# Autodesk Inventor assembly: printer_larger
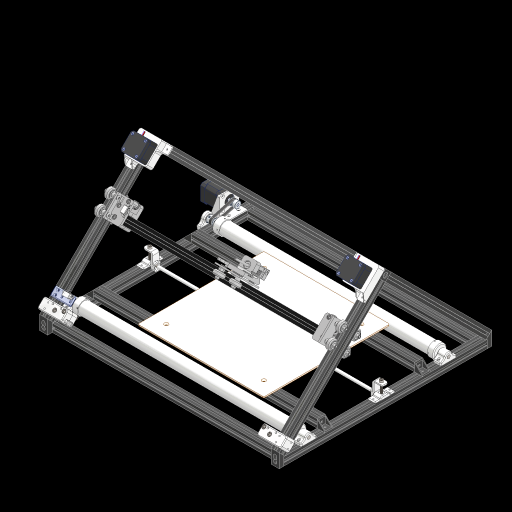
[picture p0: Inventor's stored thumbnail of the model, 512x512]
Saved by Autodesk Inventor 2023 (Build 270158000, 158)
## iProperties
Created: 2021-08-14
Part Number: printer_larger
Description: STEP AP214
Document SubType Name: Assembly
Designer: tandu
Sending System: SolidWorks 2020
Preprocessor: SwSTEP 2.0
Title: printer_larger.STEP
Revision Number: ANY
## Documents named in this file (38)
- C:\Users\tandu\Documents\GrabCAD\Custom Conveyor Belt 3D Printer\V1\Assembly.iam
- C:\Users\tandu\Documents\GrabCAD\Custom Conveyor Belt 3D Printer\V1\Parts\Frame\printer_largeeeFrame.iam
- C:\Users\tandu\Documents\GrabCAD\Custom Conveyor Belt 3D Printer\V1\Parts\printer_largeeeNEMA17_17HS19-2004S1_Stepperonline___ _________.ipt
- C:\Users\tandu\Documents\GrabCAD\Custom Conveyor Belt 3D Printer\V1\Parts\printer_largeeetensioner_mount.ipt
- C:\Users\tandu\Documents\GrabCAD\Custom Conveyor Belt 3D Printer\V1\Parts\printer_largeee5mm_roller_shaft.ipt
- C:\Users\tandu\Documents\GrabCAD\Custom Conveyor Belt 3D Printer\V1\Parts\printer_largeee330mm_cf_tube_thin.ipt
- C:\Users\tandu\Documents\GrabCAD\Custom Conveyor Belt 3D Printer\V1\Parts\printer_largeee605_bearing.ipt
- C:\Users\tandu\Documents\GrabCAD\Custom Conveyor Belt 3D Printer\V1\Parts\printer_largeeetube_mount_motor_side.ipt
- C:\Users\tandu\Documents\GrabCAD\Custom Conveyor Belt 3D Printer\V1\Parts\printer_largeeeGT2_20T_____________1.ipt
- C:\Users\tandu\Documents\GrabCAD\Custom Conveyor Belt 3D Printer\V1\Parts\printer_largeeeflange_coupling.ipt
- C:\Users\tandu\Documents\GrabCAD\Custom Conveyor Belt 3D Printer\V1\Parts\printer_largeeetube_holder_motor_side.ipt
- C:\Users\tandu\Documents\GrabCAD\Custom Conveyor Belt 3D Printer\V1\Parts\printer_largeeebelt_motor_mount.ipt
- C:\Users\tandu\Documents\GrabCAD\Custom Conveyor Belt 3D Printer\V1\Parts\printer_largeee330mm_cf_tube.ipt
- C:\Users\tandu\Documents\GrabCAD\Custom Conveyor Belt 3D Printer\V1\Parts\Build Plate\printer_largeeebed_mount_bracket.ipt
- C:\Users\tandu\Documents\GrabCAD\Custom Conveyor Belt 3D Printer\V1\Parts\printer_largeeetube_holder.ipt
- C:\Users\tandu\Documents\GrabCAD\Custom Conveyor Belt 3D Printer\V1\Parts\printer_largeeetube_mount.ipt
- C:\Users\tandu\Documents\GrabCAD\Custom Conveyor Belt 3D Printer\V1\Parts\printer_largeeeroller_rod.ipt
- C:\Users\tandu\Documents\GrabCAD\Custom Conveyor Belt 3D Printer\V1\Parts\printer_largeeeramp_mount.ipt
- C:\Users\tandu\Documents\GrabCAD\Custom Conveyor Belt 3D Printer\V1\Parts\Build Plate\printer_largeeebed_Predeterminado.ipt
- C:\Users\tandu\Documents\GrabCAD\Custom Conveyor Belt 3D Printer\V1\Parts\printer_largeeeBelt2-2987^printer_larger.ipt
- C:\Users\tandu\Documents\GrabCAD\Custom Conveyor Belt 3D Printer\V1\Parts\printer_largeeeF695 Bearing.step.ipt
- C:\Users\tandu\Documents\GrabCAD\Custom Conveyor Belt 3D Printer\V1\Parts\printer_largeeeleft_motor_mount.ipt
- C:\Users\tandu\Documents\GrabCAD\Custom Conveyor Belt 3D Printer\V1\Parts\printer_largeeeM5x40.ipt
- C:\Users\tandu\Documents\GrabCAD\Custom Conveyor Belt 3D Printer\V1\Parts\printer_largeeeright_motor_mount.ipt
- C:\Users\tandu\Documents\GrabCAD\Custom Conveyor Belt 3D Printer\V1\Parts\Gantry (Includes extruder folder)\printer_largeeegantry_idler_left.ipt
- C:\Users\tandu\Documents\GrabCAD\Custom Conveyor Belt 3D Printer\V1\Parts\Gantry (Includes extruder folder)\printer_largeeegantry_idler_right.ipt
- C:\Users\tandu\Documents\GrabCAD\Custom Conveyor Belt 3D Printer\V1\Parts\Gantry (Includes extruder folder)\printer_largeeegantry_idler_left_top.ipt
- C:\Users\tandu\Documents\GrabCAD\Custom Conveyor Belt 3D Printer\V1\Parts\Gantry (Includes extruder folder)\printer_largeeegantry_idler_right_top.ipt
- C:\Users\tandu\Documents\GrabCAD\Custom Conveyor Belt 3D Printer\V1\Parts\printer_largeeetensioner_mount_mount.ipt
- C:\Users\tandu\Documents\GrabCAD\Custom Conveyor Belt 3D Printer\V1\Parts\printer_largeeeM5x30.ipt
- C:\Users\tandu\Documents\GrabCAD\Custom Conveyor Belt 3D Printer\V1\Parts\printer_largeeey_switch_mount.ipt
- C:\Users\tandu\Documents\GrabCAD\Custom Conveyor Belt 3D Printer\V1\Parts\printer_largeeelimit_switch_cover_y.ipt
- C:\Users\tandu\Documents\GrabCAD\Custom Conveyor Belt 3D Printer\V1\Parts\printer_largeeeMicroswitch2.step_1.iam
- C:\Users\tandu\Documents\GrabCAD\Custom Conveyor Belt 3D Printer\V1\Parts\printer_largeeebearing_spacer.ipt
- C:\Users\tandu\Documents\GrabCAD\Custom Conveyor Belt 3D Printer\V1\Parts\Gantry (Includes extruder folder)\LeftGantryMount.iam
- C:\Users\tandu\Documents\GrabCAD\Custom Conveyor Belt 3D Printer\V1\Parts\Gantry (Includes extruder folder)\RightGantryMount.iam
- C:\Users\tandu\Documents\GrabCAD\Custom Conveyor Belt 3D Printer\V1\Parts\Gantry (Includes extruder folder)\Extruder\RollerVersionExtruder.iam
- C:\Users\tandu\Documents\GrabCAD\Custom Conveyor Belt 3D Printer\V1\Parts\Frame\Width Extrusion.ipt
## Components (70 placed, 69 different names)
1. Frame_1 [sub-assembly] — Tangent:1, Tangent:2, Mate:15, Angle:1, Symmetry:1, Flush:18, Mate:18, Flush:19, Mate:19, Flush:20, Flush:21, Mate:20, Mate:21, Mate:22, Mate:23, Flush:22, Flush:23, Mate:28, Mate:32, Flush:24, Flush:25, Mate:33, Mate:34, Flush:36, Flush:38, Mate:35, Angle:2, Mate:37, Mate:38, Mate:40, Flush:41, Angle:3, Mate:41, Flush:42, Mate:43, Flush:44, Mate:48, Flush:45, Flush:46, Flush:47, Mate:53, Mate:54, Mate:55, Mate:56, Mate:57, Flush:51, Flush:52, Mate:58
2. ramp_mount_34 — Flush:52, Mate:58
3. ramp_mount_35 — Mate:57, Flush:51
4. bearing_spacer_96 — Insert:32, Insert:33
5. bearing_spacer_95 — Insert:39, Insert:40
6. F695 Bearing.step_44 — Insert:33, Insert:34
7. F695 Bearing.step_45 — Insert:34
8. gantry_idler_left_59 — Insert:37, Flush:48
9. gantry_idler_right_60 — Insert:45, Flush:50
10. F695 Bearing.step_61 — Insert:40, Insert:41
11. F695 Bearing.step_62 — Insert:41
12. F695 Bearing.step_63 — Insert:38, Insert:39
13. F695 Bearing.step_64 — Insert:31, Insert:32
14. F695 Bearing.step_65 — Insert:30, Insert:31
15. F695 Bearing.step_66 — Insert:38, Insert:42
16. gantry_idler_left_top_71 — Flush:47, Mate:53, Mate:54, Insert:30, Insert:35, Insert:36, Insert:37, Flush:48, Flush:49
17. gantry_idler_right_top_72 — Flush:49, Mate:55, Mate:56, Insert:42, Insert:43, Insert:44, Insert:45, Flush:50
18. M5x40_76 — Insert:36
19. M5x40_80 — Insert:35
20. M5x40_81 — Insert:44
21. M5x40_82 — Insert:43
22. LeftGantryMount:1 [sub-assembly] — Tangent:1, Tangent:2, Mate:9, Mate:10, Mate:11, Flush:17
23. RightGantryMount:1 [sub-assembly] — Mate:12, Mate:13, Mate:14
24. RollerVersionExtruder:1 [sub-assembly] — Mate:9, Mate:10, Mate:11, Mate:12, Mate:13, Mate:14
25. y_switch_mount_91 — Mate:48, Flush:45, Mate:49, Insert:28, Insert:29, Mate:51, Flush:46
26. limit_switch_cover_y_92 — Mate:49, Insert:28, Insert:29, Mate:50, Mate:52
27. Microswitch2.step_93 [sub-assembly] — Mate:50, Mate:51, Mate:52
28. flange_coupling_14 — Insert:11, Mate:25, Mate:26
29. 5mm_roller_shaft_13 — Mate:24
30. 605_bearing_9 — Insert:9, Insert:10
31. GT2_20T_____________1_11 — Insert:10, Insert:11, Mate:30, Mate:31
32. 5mm_roller_shaft_5 — Insert:22
33. 5mm_roller_shaft_6 — Insert:21
34. roller_rod_33 — Insert:14, Mate:27
35. roller_rod_30 — Insert:26, Mate:44
36. roller_rod_28 — Flush:43, Mate:42
37. tube_holder_25 — Insert:24, Insert:25
38. bed_Predeterminado_36
39. tensioner_mount_4 — Insert:19, Mate:36, Angle:2, Insert:20, Insert:22
40. tensioner_mount_7 — Insert:21, Insert:23, Angle:3
41. 330mm_cf_tube_thin_8 — Insert:20
42. tube_mount_motor_side_10 — Mate:23, Flush:22, Insert:9, Mate:24
43. tube_holder_motor_side_15 — Mate:25, Mate:26, Insert:12
44. 330mm_cf_tube_19 — Insert:25, Insert:27
45. 330mm_cf_tube_20 — Insert:12, Insert:13
46. tube_holder_26 — Insert:27, Mate:44
47. tube_mount_27 — Mate:41, Flush:42, Flush:43, Mate:42, Insert:24
48. tube_mount_29 — Insert:26, Mate:43, Flush:44, Mate:45, Mate:47
49. tube_holder_31 — Insert:13, Mate:27
50. tube_mount_32 — Insert:14, Flush:23, Mate:28, Mate:45
51. tensioner_mount_mount_85 — Mate:38, Flush:40, Mate:39, Mate:40, Flush:41
52. M5x30_86 — Flush:40, Mate:39, Insert:23
53. tensioner_mount_mount_87 — Flush:38, Mate:35, Mate:36, Mate:37, Flush:39
54. M5x30_88 — Insert:19, Flush:39
55. NEMA17_17HS19-2004S1_Stepperonline___ __________2 — Insert:6, Insert:7, Insert:8
56. NEMA17_17HS19-2004S1_Stepperonline___ __________39 — Mate:16, Mate:17, Insert:1, Insert:2
57. NEMA17_17HS19-2004S1_Stepperonline___ __________40 — Insert:3, Insert:4, Insert:5
58. belt_motor_mount_16 — Mate:20, Mate:21, Mate:22, Insert:6, Insert:7
59. left_motor_mount_53 — Insert:3, Mate:19, Flush:20, Flush:21, Insert:5
60. right_motor_mount_58 — Insert:1, Insert:2, Flush:18, Mate:18, Flush:19
61. GT2_20T_____________1_12 — Insert:8, Mate:29
62. Belt2-2987^printer_larger_38 — Mate:29, Mate:30, Mate:31
63. GT2_20T_____________1_41 — Mate:16, Mate:17
64. GT2_20T_____________1_42 — Insert:4
65. width extrusion:1 — Insert:15, Insert:16, Mate:46
66. width extrusion:2 — Insert:17, Flush:37, Insert:18, Mate:46
67. bed_mount_bracket_21 — Mate:32, Flush:24, Insert:15
68. bed_mount_bracket_22 — Mate:34, Flush:36, Insert:17, Flush:37
69. bed_mount_bracket_23 — Flush:25, Mate:33, Insert:18, Mate:47
70. bed_mount_bracket_24 — Insert:16
## Relationships (127: Mate 50, Insert 45, Flush 26, Angle 3, Tangent 2, Symmetry 1)
- Tangent:1: Frame_1 ↔ LeftGantryMount:1
- Tangent:2: Frame_1 ↔ LeftGantryMount:1
- Mate:9: LeftGantryMount:1 ↔ RollerVersionExtruder:1
- Mate:10: LeftGantryMount:1 ↔ RollerVersionExtruder:1
- Mate:11: LeftGantryMount:1 ↔ RollerVersionExtruder:1
- Mate:12: RightGantryMount:1 ↔ RollerVersionExtruder:1
- Mate:13: RightGantryMount:1 ↔ RollerVersionExtruder:1
- Mate:14: RightGantryMount:1 ↔ RollerVersionExtruder:1
- Mate:15: Frame_1
- Angle:1 (0 deg): Frame_1
- Symmetry:1: Frame_1
- Flush:17: LeftGantryMount:1
- Mate:16 (6 mm): NEMA17_17HS19-2004S1_Stepperonline___ __________39 ↔ GT2_20T_____________1_41
- Mate:17: NEMA17_17HS19-2004S1_Stepperonline___ __________39 ↔ GT2_20T_____________1_41
- Insert:1: NEMA17_17HS19-2004S1_Stepperonline___ __________39 ↔ right_motor_mount_58
- Insert:2: NEMA17_17HS19-2004S1_Stepperonline___ __________39 ↔ right_motor_mount_58
- Flush:18: Frame_1 ↔ right_motor_mount_58
- Mate:18: Frame_1 ↔ right_motor_mount_58
- Flush:19: Frame_1 ↔ right_motor_mount_58
- Insert:3: NEMA17_17HS19-2004S1_Stepperonline___ __________40 ↔ left_motor_mount_53
- Insert:4 (6 mm): NEMA17_17HS19-2004S1_Stepperonline___ __________40 ↔ GT2_20T_____________1_42
- Mate:19: Frame_1 ↔ left_motor_mount_53
- Flush:20: Frame_1 ↔ left_motor_mount_53
- Flush:21: Frame_1 ↔ left_motor_mount_53
- Insert:5: NEMA17_17HS19-2004S1_Stepperonline___ __________40 ↔ left_motor_mount_53
- Mate:20: Frame_1 ↔ belt_motor_mount_16
- Mate:21: Frame_1 ↔ belt_motor_mount_16
- Mate:22: Frame_1 ↔ belt_motor_mount_16
- Insert:6: NEMA17_17HS19-2004S1_Stepperonline___ __________2 ↔ belt_motor_mount_16
- Insert:7: NEMA17_17HS19-2004S1_Stepperonline___ __________2 ↔ belt_motor_mount_16
- Mate:23: Frame_1 ↔ tube_mount_motor_side_10
- Flush:22: Frame_1 ↔ tube_mount_motor_side_10
- Insert:8 (6 mm): NEMA17_17HS19-2004S1_Stepperonline___ __________2 ↔ GT2_20T_____________1_12
- Insert:9: 605_bearing_9 ↔ tube_mount_motor_side_10
- Insert:10 (1.6 mm): 605_bearing_9 ↔ GT2_20T_____________1_11
- Mate:24: 5mm_roller_shaft_13 ↔ tube_mount_motor_side_10
- Insert:11 (2.5 mm): flange_coupling_14 ↔ GT2_20T_____________1_11
- Mate:25: flange_coupling_14 ↔ tube_holder_motor_side_15
- Mate:26: flange_coupling_14 ↔ tube_holder_motor_side_15
- Insert:12: tube_holder_motor_side_15 ↔ 330mm_cf_tube_20
- Insert:13: 330mm_cf_tube_20 ↔ tube_holder_31
- Insert:14: roller_rod_33 ↔ tube_mount_32
- Mate:27: roller_rod_33 ↔ tube_holder_31
- Flush:23: Frame_1 ↔ tube_mount_32
- Mate:28: Frame_1 ↔ tube_mount_32
- Mate:29: GT2_20T_____________1_12 ↔ Belt2-2987^printer_larger_38
- Mate:30: GT2_20T_____________1_11 ↔ Belt2-2987^printer_larger_38
- Mate:31: GT2_20T_____________1_11 ↔ Belt2-2987^printer_larger_38
- Mate:32: Frame_1 ↔ bed_mount_bracket_21
- Flush:24: Frame_1 ↔ bed_mount_bracket_21
- Insert:15: width extrusion:1 ↔ bed_mount_bracket_21
- Insert:16: width extrusion:1 ↔ bed_mount_bracket_24
- Flush:25: Frame_1 ↔ bed_mount_bracket_23
- Mate:33: Frame_1 ↔ bed_mount_bracket_23
- Mate:34: Frame_1 ↔ bed_mount_bracket_22
- Flush:36: Frame_1 ↔ bed_mount_bracket_22
- Insert:17: width extrusion:2 ↔ bed_mount_bracket_22
- Flush:37: width extrusion:2 ↔ bed_mount_bracket_22
- Insert:18: width extrusion:2 ↔ bed_mount_bracket_23
- Flush:38: Frame_1 ↔ tensioner_mount_mount_87
- Mate:35: Frame_1 ↔ tensioner_mount_mount_87
- Insert:19: tensioner_mount_4 ↔ M5x30_88
- Mate:36: tensioner_mount_4 ↔ tensioner_mount_mount_87
- Angle:2 (180 deg): Frame_1 ↔ tensioner_mount_4
- Mate:37: Frame_1 ↔ tensioner_mount_mount_87
- Flush:39: tensioner_mount_mount_87 ↔ M5x30_88
- Insert:20 (1 mm): tensioner_mount_4 ↔ 330mm_cf_tube_thin_8
- Insert:21: 5mm_roller_shaft_6 ↔ tensioner_mount_7
- Insert:22: 5mm_roller_shaft_5 ↔ tensioner_mount_4
- Mate:38: Frame_1 ↔ tensioner_mount_mount_85
- Flush:40: tensioner_mount_mount_85 ↔ M5x30_86
- Mate:39: tensioner_mount_mount_85 ↔ M5x30_86
- Mate:40: Frame_1 ↔ tensioner_mount_mount_85
- Flush:41: Frame_1 ↔ tensioner_mount_mount_85
- Insert:23: tensioner_mount_7 ↔ M5x30_86
- Angle:3 (180 deg): Frame_1 ↔ tensioner_mount_7
- Mate:41: Frame_1 ↔ tube_mount_27
- Flush:42: Frame_1 ↔ tube_mount_27
- Flush:43: roller_rod_28 ↔ tube_mount_27
- Mate:42: roller_rod_28 ↔ tube_mount_27
- Insert:24 (2 mm): tube_holder_25 ↔ tube_mount_27
- Insert:25: tube_holder_25 ↔ 330mm_cf_tube_19
- Insert:26: roller_rod_30 ↔ tube_mount_29
- Insert:27: 330mm_cf_tube_19 ↔ tube_holder_26
- Mate:43: Frame_1 ↔ tube_mount_29
- Flush:44: Frame_1 ↔ tube_mount_29
- Mate:44: roller_rod_30 ↔ tube_holder_26
- Mate:45 (304 mm): tube_mount_29 ↔ tube_mount_32
- Mate:46 (220 mm): width extrusion:1 ↔ width extrusion:2
- Mate:47 (20 mm): tube_mount_29 ↔ bed_mount_bracket_23
- Mate:48: Frame_1 ↔ y_switch_mount_91
- Flush:45: Frame_1 ↔ y_switch_mount_91
- Mate:49: y_switch_mount_91 ↔ limit_switch_cover_y_92
- Insert:28: y_switch_mount_91 ↔ limit_switch_cover_y_92
- Insert:29: y_switch_mount_91 ↔ limit_switch_cover_y_92
- Mate:50: limit_switch_cover_y_92 ↔ Microswitch2.step_93
- Mate:51: y_switch_mount_91 ↔ Microswitch2.step_93
- Mate:52: limit_switch_cover_y_92 ↔ Microswitch2.step_93
- Flush:46 (38 mm): Frame_1 ↔ y_switch_mount_91
- Flush:47 (7 mm): Frame_1 ↔ gantry_idler_left_top_71
- Mate:53: Frame_1 ↔ gantry_idler_left_top_71
- Mate:54: Frame_1 ↔ gantry_idler_left_top_71
- Insert:30: F695 Bearing.step_65 ↔ gantry_idler_left_top_71
- Insert:31: F695 Bearing.step_64 ↔ F695 Bearing.step_65
- Insert:32 (0.2 mm): bearing_spacer_96 ↔ F695 Bearing.step_64
- Insert:33: bearing_spacer_96 ↔ F695 Bearing.step_44
- Insert:34: F695 Bearing.step_44 ↔ F695 Bearing.step_45
- Insert:35: gantry_idler_left_top_71 ↔ M5x40_80
- Insert:36: gantry_idler_left_top_71 ↔ M5x40_76
- Insert:37: gantry_idler_left_59 ↔ gantry_idler_left_top_71
- Flush:48: gantry_idler_left_59 ↔ gantry_idler_left_top_71
- Flush:49: gantry_idler_left_top_71 ↔ gantry_idler_right_top_72
- Mate:55: Frame_1 ↔ gantry_idler_right_top_72
- Mate:56: Frame_1 ↔ gantry_idler_right_top_72
- Insert:38: F695 Bearing.step_63 ↔ F695 Bearing.step_66
- Insert:39 (0.2 mm): bearing_spacer_95 ↔ F695 Bearing.step_63
- Insert:40: bearing_spacer_95 ↔ F695 Bearing.step_61
- Insert:41: F695 Bearing.step_61 ↔ F695 Bearing.step_62
- Insert:42: F695 Bearing.step_66 ↔ gantry_idler_right_top_72
- Insert:43: gantry_idler_right_top_72 ↔ M5x40_82
- Insert:44: gantry_idler_right_top_72 ↔ M5x40_81
- Insert:45: gantry_idler_right_60 ↔ gantry_idler_right_top_72
- Flush:50: gantry_idler_right_60 ↔ gantry_idler_right_top_72
- Mate:57: Frame_1 ↔ ramp_mount_35
- Flush:51: Frame_1 ↔ ramp_mount_35
- Flush:52: Frame_1 ↔ ramp_mount_34
- Mate:58: Frame_1 ↔ ramp_mount_34
